# Autodesk Inventor assembly: bellows-clamped-on-bearings
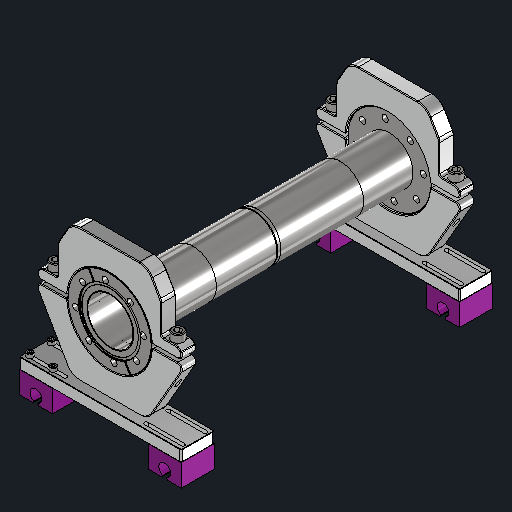
[picture p0: Inventor's stored thumbnail of the model, 512x512]
Saved by Autodesk Inventor 2027.1 (Build 311270010, 270A)
## iProperties
Created: 2026-10-08
Part Number: bellows-clamped-on-bearings
Document SubType Name: Assembly
Designer: queezz
Author: queezz
## Documents named in this file (8)
- C:\Users\queezz\Dropbox\Drawings\pihti-cad\bellows-probe\bellows-clamped-on-bearings.iam
- C:\Users\queezz\Dropbox\Drawings\pihti-cad\bellows-probe\flange-camp-114.ipt
- C:\Users\queezz\Dropbox\Drawings\pihti-cad\bellows-probe\bellows_flange.ipt
- C:\Users\queezz\Dropbox\Drawings\pihti-cad\bellows-probe\linearbearing.ipt
- C:\Users\queezz\Dropbox\Drawings\pihti-cad\bellows-probe\instead-of-bellows.ipt
- C:\Users\queezz\Dropbox\Drawings\pihti-cad\bellows-probe\clamp-foot.ipt
- C:\Users\queezz\Dropbox\Drawings\pihti-cad\ContentCenter\Fastners\M5x20-SHCS.ipt
- C:\Users\queezz\Documents\Inventor\Content Center Files\R2027\en-US\AS 1420\AS 1420 - 1973 - M10 x 30.ipt
## Components (21 placed, 7 different names)
1. flange-camp-114:1
2. flange-camp-114:2
3. bellows_flange:1
4. bellows_flange:2
5. linearbearing:1 — Mate:13, Flush:12
6. linearbearing:2 — Mate:14, Flush:10
7. linearbearing:3 — Mate:14, Flush:11
8. linearbearing:4 — Mate:13, Flush:13
9. instead-of-bellows:1
10. instead-of-bellows:2
11. clamp-foot:1 — Flush:11, Flush:12
12. clamp-foot:2 — Flush:10, Flush:13
13. instead-of-bellows:3
14. instead-of-bellows:4
15. AS 1420 - Metric M10 x 30:4
16. AS 1420 - Metric M10 x 30:3
17. AS 1420 - Metric M10 x 30:2
18. AS 1420 - Metric M10 x 30:1
19. AS 1420 - Metric M5 x 20:3
20. AS 1420 - Metric M5 x 20:2
21. AS 1420 - Metric M5 x 20:1
## Relationships (38: Mate 14, Flush 13, WeldJoint 10, RevoluteJoint 1)
- [Flush]: linearbearing:2 ↔ linearbearing:4
- [Flush]: linearbearing:1 ↔ linearbearing:3
- [Flush]: linearbearing:2 ↔ linearbearing:4
- [WeldJoint]: bellows_flange:2 ↔ instead-of-bellows:1
- [WeldJoint]: bellows_flange:1 ↔ instead-of-bellows:2
- [Mate]: instead-of-bellows:1 ↔ instead-of-bellows:2
- [Mate]: linearbearing:3 ↔ clamp-foot:1
- [Flush]: flange-camp-114:1 ↔ clamp-foot:2
- [Mate]: flange-camp-114:1 ↔ clamp-foot:2
- [Flush]: linearbearing:4 ↔ clamp-foot:2
- [Flush]: linearbearing:4 ↔ clamp-foot:2
- [Mate]: flange-camp-114:1 ↔ clamp-foot:2
- [Mate] (-650 mm): bellows_flange:1 ↔ bellows_flange:2
- [Mate]: instead-of-bellows:1 ↔ instead-of-bellows:4
- [Mate]: instead-of-bellows:2 ↔ instead-of-bellows:3
- [Mate]: instead-of-bellows:2 ↔ instead-of-bellows:3
- [Mate] (-200 mm): instead-of-bellows:1 ↔ instead-of-bellows:4
- [Mate]: instead-of-bellows:3 ↔ instead-of-bellows:4
- [Mate]: flange-camp-114:2 ↔ clamp-foot:1
- [Mate]: flange-camp-114:2 ↔ clamp-foot:1
- [Flush]: flange-camp-114:2 ↔ clamp-foot:1
- [Flush]: linearbearing:1 ↔ clamp-foot:1
- [Flush]: linearbearing:3 ↔ clamp-foot:1
- [WeldJoint]: flange-camp-114:1 ↔ bellows_flange:2
- [WeldJoint]: flange-camp-114:2 ↔ bellows_flange:1
- Mate:13: linearbearing:1 ↔ linearbearing:4
- Mate:14: linearbearing:2 ↔ linearbearing:3
- Flush:10: linearbearing:2 ↔ clamp-foot:2
- Flush:11: linearbearing:3 ↔ clamp-foot:1
- Flush:12: linearbearing:1 ↔ clamp-foot:1
- Flush:13: linearbearing:4 ↔ clamp-foot:2
- [WeldJoint] (15 mm): linearbearing:3 ↔ AS 1420 - Metric M5 x 20:1
- [WeldJoint] (15 mm): linearbearing:3 ↔ AS 1420 - Metric M5 x 20:2
- [RevoluteJoint] (15 mm): linearbearing:3 ↔ AS 1420 - Metric M5 x 20:3
- [WeldJoint]: flange-camp-114:2 ↔ AS 1420 - Metric M10 x 30:1
- [WeldJoint]: flange-camp-114:2 ↔ AS 1420 - Metric M10 x 30:2
- [WeldJoint]: flange-camp-114:1 ↔ AS 1420 - Metric M10 x 30:3
- [WeldJoint]: flange-camp-114:1 ↔ AS 1420 - Metric M10 x 30:4
## Named parameters: d24_d26 = 0 mm
